# Autodesk Inventor assembly: 組合檔
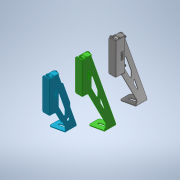
[picture p0: Inventor's stored thumbnail of the model, 180x180]
Saved by Autodesk Inventor 2020 (Build 240168000, 168)
## iProperties
Created: 2015-11-28
Part Number: 組合檔
Document SubType Name: Assembly
Designer: 設計製圖
Author: 設計製圖
## Documents named in this file (4)
- D:\資料庫\設計-3D Project\【May club 】\得利卡-車頂燈架\模型、圖面\長、短-對照.iam
- D:\資料庫\設計-3D Project\【May club 】\得利卡-車頂燈架\模型、圖面\短-車頂燈架-組合(#11.02).iam
- D:\資料庫\設計-3D Project\【May club 】\得利卡-車頂燈架\模型、圖面\old\長-車頂燈架-組合(#11.02).iam
- D:\資料庫\設計-3D Project\【May club 】\得利卡-車頂燈架\模型、圖面\版本-吊架-長(#11.26)\長-車頂燈架-組合(#11.26).iam
## Components (3 placed, 3 different names)
1. 短-車頂燈架-組合(#11.02):1 [sub-assembly] — 齊平:1, 齊平:2
2. 長-車頂燈架-組合(#11.02):1 [sub-assembly] — 齊平:1, 齊平:2, 齊平:3, 齊平:4
3. 長-車頂燈架-組合(#11.26):1 [sub-assembly] — 齊平:3, 齊平:4
## Relationships (4: Flush 4)
- 齊平:1 [Flush]: 短-車頂燈架-組合(#11.02):1 ↔ 長-車頂燈架-組合(#11.02):1
- 齊平:2 [Flush]: 短-車頂燈架-組合(#11.02):1 ↔ 長-車頂燈架-組合(#11.02):1
- 齊平:3 [Flush]: 長-車頂燈架-組合(#11.02):1 ↔ 長-車頂燈架-組合(#11.26):1
- 齊平:4 [Flush]: 長-車頂燈架-組合(#11.02):1 ↔ 長-車頂燈架-組合(#11.26):1
